# Autodesk Inventor assembly: Quad Assy
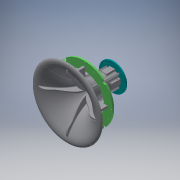
[picture p0: Inventor's stored thumbnail of the model, 180x180]
Saved by Autodesk Inventor 2016 SP1 (Build 200210100, 210)
## iProperties
Created: 2015-10-31
Part Number: Quad Assy
Description: STEP AP214
Document SubType Name: Assembly
Designer: Dave
Sending System: SolidWorks 2003240
Preprocessor: SwSTEP 2.0
Title: Quad Assy.STEP
Revision Number: ANY
## Documents named in this file (10)
- C:\Users\ddeboer\Desktop\leuschner-cad\Quad Assy.iam
- C:\Users\ddeboer\Desktop\leuschner-cad\connector.ipt
- C:\Users\ddeboer\Desktop\leuschner-cad\1.15 Quadrent 1.ipt
- C:\Users\ddeboer\Desktop\leuschner-cad\Berkeley ring.ipt
- C:\Users\ddeboer\Desktop\leuschner-cad\Mtg Ring.ipt
- C:\Users\ddeboer\Desktop\leuschner-cad\1.15 Quadrent 1_Default .437.ipt
- C:\Users\ddeboer\Desktop\leuschner-cad\Horn Base.ipt
- C:\Users\ddeboer\Desktop\leuschner-cad\1.15 Quadrent 1_Opposite.ipt
- C:\Users\ddeboer\Desktop\leuschner-cad\1.15 Quadrent 1_Opposide 437.ipt
- C:\Users\ddeboer\Desktop\leuschner-cad\pin.ipt
## Components (13 placed, 13 different names)
1. connector_1
2. 1.15 Quadrent 1_2 — Mate:1
3. Berkeley ring_3
4. Mtg Ring_4 — Mate:1, Insert:1
5. Berkeley ring_5
6. 1.15 Quadrent 1_Default .437_6
7. Horn Base_7
8. Berkeley ring_8
9. 1.15 Quadrent 1_Opposite_9
10. Berkeley ring_10
11. connector_11
12. 1.15 Quadrent 1_Opposide 437_12 — Insert:1
13. pin_13
## Relationships (2: Mate 1, Insert 1)
- Mate:1: 1.15 Quadrent 1_2 ↔ Mtg Ring_4
- Insert:1: Mtg Ring_4 ↔ 1.15 Quadrent 1_Opposide 437_12
